# Autodesk Inventor assembly: Nema23MetGearbox
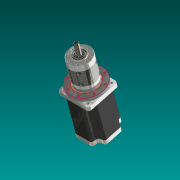
[picture p0: Inventor's stored thumbnail of the model, 180x180]
Saved by Autodesk Inventor 2020.3 (Build 243373000, 373)
## iProperties
Created: 2020-05-18
Part Number: Nema23MetGearbox
Document SubType Name: Assembly
Designer: Svend
Author: Svend
## Documents named in this file (6)
- C:\Users\Svend\OneDrive\Documents\GitHub\BeerMinder\3D-model\subAssembly\Nema23MetGearbox.iam
- C:\Users\Svend\OneDrive\Documents\GitHub\BeerMinder\3D-model\gearbox\gearbox.iam
- C:\Users\Svend\OneDrive\Documents\GitHub\BeerMinder\3D-model\stepper motors\Nema 23 High toque.ipt
- C:\Users\Svend\OneDrive\Documents\GitHub\BeerMinder\3D-model\subAssembly\koppelstukje nema23.ipt
- C:\Users\Svend\OneDrive\Documents\GitHub\BeerMinder\3D-model\subAssembly\as gearbox.ipt
- C:\Users\Svend\OneDrive\Documents\GitHub\BeerMinder\3D-model\bearings\slewbearing\slewbearing nema23\Slew Bearing nema23.iam
## Components (5 placed, 5 different names)
1. gearbox:1 [sub-assembly] — Mate:1, Mate:3, Mate:7
2. Nema 23 High toque:1 — Mate:1, Mate:2, Mate:6, Angle:1
3. koppelstukje nema23:1 — Mate:2, Mate:4, Flush:2, Mate:5
4. as gearbox:1 — Mate:3, Mate:4, Flush:2
5. Slew Bearing nema23:1 [sub-assembly] — Mate:5, Mate:6, Mate:7, Angle:1
## Relationships (9: Mate 7, Flush 1, Angle 1)
- Mate:1: gearbox:1 ↔ Nema 23 High toque:1
- Mate:2: Nema 23 High toque:1 ↔ koppelstukje nema23:1
- Mate:3: gearbox:1 ↔ as gearbox:1
- Mate:4: koppelstukje nema23:1 ↔ as gearbox:1
- Flush:2 (-5 mm): koppelstukje nema23:1 ↔ as gearbox:1
- Mate:5: koppelstukje nema23:1 ↔ Slew Bearing nema23:1
- Mate:6: Nema 23 High toque:1 ↔ Slew Bearing nema23:1
- Mate:7: gearbox:1 ↔ Slew Bearing nema23:1
- Angle:1 (22.5 deg): Nema 23 High toque:1 ↔ Slew Bearing nema23:1
